# Autodesk Inventor assembly: hoop2_cog
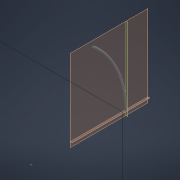
[picture p0: Inventor's stored thumbnail of the model, 180x180]
Saved by Autodesk Inventor 2021 (Build 250183000, 183)
## iProperties
Created: 2021-06-13
Part Number: hoop2_cog
Document SubType Name: Assembly
Designer: Watchdog
Mass: 3439.74 g
Surface Area: 2881.77 cm^2
Volume: 438.183 cm^3
Density: 7.85 g/cm^3
Author: Watchdog
## Documents named in this file (2)
- C:\Users\Watchdog\OneDrive - Flinders\Advn Mech Design Shared\6_Development\2_Design\inventor\hoop_slider\validationfiles\hoop2_cog.iam
- C:\Users\Watchdog\OneDrive - Flinders\Advn Mech Design Shared\6_Development\2_Design\inventor\hoop_slider\medium_hoop.ipt
## Components (1 placed, 1 different names)
1. medium_hoop:1 — Flush:1
## Relationships (2: Flush 1, Angle 1)
- Flush:1: medium_hoop:1
- Angle:1 (-42 deg)
